# Autodesk Inventor assembly: New Final Leg Assembly
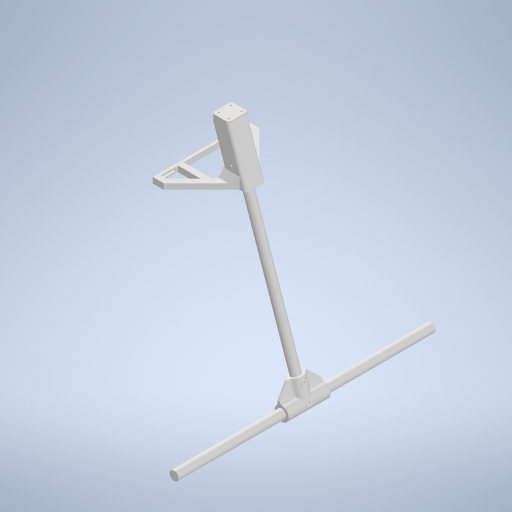
[picture p0: Inventor's stored thumbnail of the model, 512x512]
Saved by Autodesk Inventor 2023 (Build 270158000, 158)
## iProperties
Created: 2023-01-21
Part Number: New Final Leg Assembly
Document SubType Name: Assembly
Designer: chase
Author: chase
## Documents named in this file (5)
- C:\Users\Administrator\Documents\GitHub\WU-Team20-AutonomousDrone\CAD\ASSEMBLY\SubAssembly - Leg SingleSide.iam
- C:\Users\Administrator\Documents\GitHub\WU-Team20-AutonomousDrone\CAD\Legs\UpperLandingLegMount - WebBrace+Shortened.ipt
- C:\Users\Administrator\Documents\GitHub\WU-Team20-AutonomousDrone\CAD\Raw Models\CarbonTube - 16ODx333mm.ipt
- C:\Users\Administrator\Documents\GitHub\WU-Team20-AutonomousDrone\CAD\Legs\LegTeeJoint - 16x16mmHoles.ipt
- C:\Users\Administrator\Documents\GitHub\WU-Team20-AutonomousDrone\CAD\Raw Models\CarbonTube - 16ODx457,2mm.ipt
## Components (4 placed, 4 different names)
1. UpperLandingLegMount - WebBrace+Shortened:1 — Insert:1
2. CarbonTube - 16ODx333mm:1 — Insert:1, Insert:2
3. LegTeeJoint - 16x16mmHoles:1 — Insert:2, Insert:3
4. CarbonTube - 16ODx457,2mm:1 — Insert:3
## Relationships (3: Insert 3)
- Insert:1: UpperLandingLegMount - WebBrace+Shortened:1 ↔ CarbonTube - 16ODx333mm:1
- Insert:2: CarbonTube - 16ODx333mm:1 ↔ LegTeeJoint - 16x16mmHoles:1
- Insert:3 (-191.1 mm): LegTeeJoint - 16x16mmHoles:1 ↔ CarbonTube - 16ODx457,2mm:1
